# Autodesk Inventor assembly: Assembly1
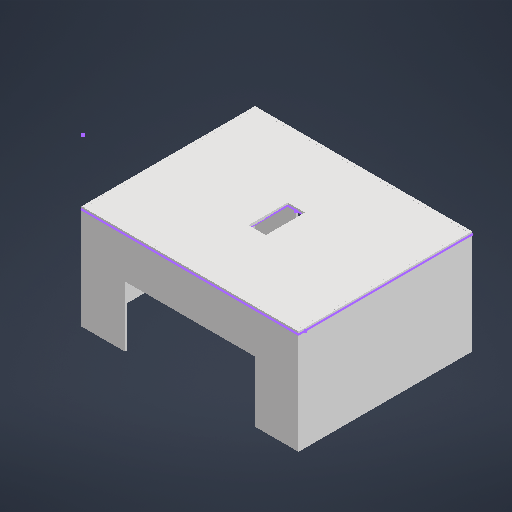
[picture p0: Inventor's stored thumbnail of the model, 512x512]
Saved by Autodesk Inventor 2027.1 (Build 311270010, 270A)
## iProperties
Created: 2026-10-07
Part Number: Assembly1
Document SubType Name: Assembly
Designer: daniel
Author: daniel
## Documents named in this file (4)
- C:\Users\danda\Desktop\Design 1\Project\CAD\box\Assembly1.iam
- C:\Users\danda\Desktop\Design 1\Project\CAD\box\Part2.ipt
- C:\Users\danda\Desktop\Design 1\Project\CAD\box\Part1.ipt
- C:\Users\danda\Desktop\Design 1\Project\CAD\box\part5.ipt
## Components (5 placed, 3 different names)
1. Part2:1 — Mate:1, Flush:1, Mate:2, Mate:6, Mate:7, Flush:3, Mate:11
2. Part1:1 — Mate:1, Flush:1, Mate:2, Mate:13
3. Part2:2 — Mate:8, Mate:9, Mate:10
4. Part1:2 — Mate:6, Mate:7, Flush:3, Mate:8, Mate:9, Mate:10, Mate:12
5. part5:1 — Mate:11, Mate:12, Mate:13
## Relationships (12: Mate 10, Flush 2)
- Mate:1: Part2:1 ↔ Part1:1
- Flush:1: Part2:1 ↔ Part1:1
- Mate:2: Part2:1 ↔ Part1:1
- Mate:6: Part2:1 ↔ Part1:2
- Mate:7: Part2:1 ↔ Part1:2
- Flush:3: Part2:1 ↔ Part1:2
- Mate:8: Part2:2 ↔ Part1:2
- Mate:9: Part2:2 ↔ Part1:2
- Mate:10: Part2:2 ↔ Part1:2
- Mate:11: Part2:1 ↔ part5:1
- Mate:12: Part1:2 ↔ part5:1
- Mate:13: Part1:1 ↔ part5:1
